# Autodesk Inventor assembly: V2-Output-.5inHex
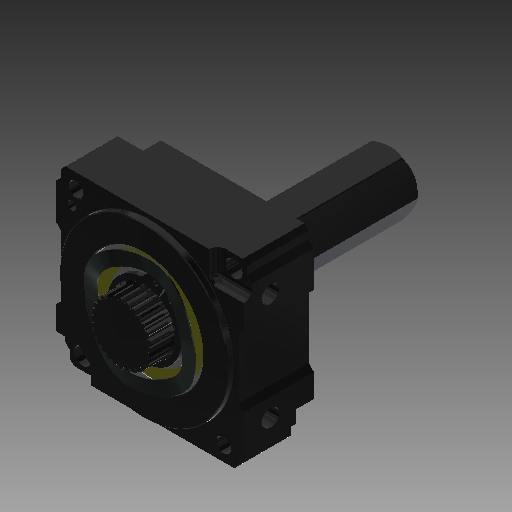
[picture p0: Inventor's stored thumbnail of the model, 512x512]
Saved by Autodesk Inventor 2023 (Build 270158000, 158)
## iProperties
Created: 2018-08-19
Part Number: V2-Output-.5inHex
Document SubType Name: Assembly
Mass: 68.0389 g
Surface Area: 166.113 cm^2
Volume: 34.5687 cm^3
Density: 1.96822 g/cm^3
## Documents named in this file (19)
- E:\Collaborative Robots\Collaborative Part Library\General Gearboxes\Planetaries\DEPRECATED Versaplanetary\V2 Stages\V2 Output Stage.iam
- E:\Collaborative Robots\Collaborative Part Library\General Gearboxes\Planetaries\DEPRECATED Versaplanetary\V2 Stages\V2 Output Housing.ipt
- E:\Collaborative Robots\Collaborative Part Library\General Gearboxes\Planetaries\DEPRECATED Versaplanetary\V2 Stages\Wave Washer.ipt
- E:\Collaborative Robots\Collaborative Part Library\General Gearboxes\Planetaries\DEPRECATED Versaplanetary\Output Shafts\VP 1-2inHex Output.ipt
- E:\Collaborative Robots\Collaborative Part Library\General Gearboxes\Planetaries\DEPRECATED Versaplanetary\V2 Stages\Retaining Ring.ipt
- E:\Collaborative Robots\Collaborative Part Library\General Gearboxes\Planetaries\DEPRECATED Versaplanetary\Output Shafts\VP 1-2inRound Output.ipt
- E:\Collaborative Robots\Collaborative Part Library\General Gearboxes\Planetaries\DEPRECATED Versaplanetary\Output Shafts\VP 3-8inHex Output.ipt
- E:\Collaborative Robots\Collaborative Part Library\General Gearboxes\Planetaries\DEPRECATED Versaplanetary\Output Shafts\VP CIM Output.ipt
- E:\Collaborative Robots\Collaborative Part Library\General Gearboxes\Planetaries\DEPRECATED Versaplanetary\Output Shafts\Universal Output shaft.ipt
- E:\Collaborative Robots\Collaborative Part Library\Power Transfer\Bearings and Bushings\Bearings\6902ZZ.ipt
- E:\Elipse 6814\Elipse Parts Library\Shaft Accessories\Bearings.ipt
- E:\Collaborative Robots\Collaborative Part Library\General Gearboxes\Planetaries\DEPRECATED Versaplanetary\VP 90 deg.ipt
- E:\Collaborative Robots\Collaborative Part Library\General Gearboxes\Planetaries\DEPRECATED Versaplanetary\Female Outputs\Universal Female Output Shaft 1_2_ Hex.ipt
- V2 Output Stage 90 deg.iam
- VP V2 Output Stage 1-2in Hex.iam
- VP V2 Output Stage 3-8in Hex.iam
- VP V2 Output Stage CIM.iam
- VP V2 Output Stage Female.iam
- VP V2 Output Stage Round.iam
## Components (12 placed, 11 different names)
1. V2 Output Housing:1 — Insert:2, Mate:2, Insert:18, Mate:3, Angle:6, Flush:7
2. 6902ZZ:1 — Insert:2, Insert:23
3. 6902ZZ:2 — Insert:18, Insert:19, Insert:20, Insert:22, Insert:24, Insert:25
4. Wave Washer:1 — Mate:2
5. Retaining Ring:1 — Angle:1, Angle:2, Angle:3, Angle:4, Angle:5, Insert:23
6. VP 1-2inHex Output:1 — Angle:1, Insert:20
7. VP 1-2inRound Output:1 — Angle:2, Insert:19
8. VP 3-8inHex Output:1 — Angle:3, Insert:22
9. VP CIM Output:1 — Angle:4, Insert:24
10. Universal Output shaft:1 — Angle:5, Insert:25, Insert:26
11. VP 90 deg:1 — Flush:8, Mate:5, Angle:7
12. Universal Female Output Shaft 1_2_ Hex:1 — Insert:26
## Relationships (21: Insert 9, Angle 7, Mate 3, Flush 2)
- Insert:2: V2 Output Housing:1 ↔ 6902ZZ:1
- Mate:2: V2 Output Housing:1 ↔ Wave Washer:1
- Angle:1 (0 deg): Retaining Ring:1 ↔ VP 1-2inHex Output:1
- Angle:2 (0 deg): Retaining Ring:1 ↔ VP 1-2inRound Output:1
- Angle:3 (0 deg): Retaining Ring:1 ↔ VP 3-8inHex Output:1
- Angle:4 (0 deg): Retaining Ring:1 ↔ VP CIM Output:1
- Angle:5 (0 deg): Retaining Ring:1 ↔ Universal Output shaft:1
- Insert:18: V2 Output Housing:1 ↔ 6902ZZ:2
- Insert:19: 6902ZZ:2 ↔ VP 1-2inRound Output:1
- Insert:20: 6902ZZ:2 ↔ VP 1-2inHex Output:1
- Insert:22: 6902ZZ:2 ↔ VP 3-8inHex Output:1
- Insert:23 (0.508 mm): 6902ZZ:1 ↔ Retaining Ring:1
- Insert:24: 6902ZZ:2 ↔ VP CIM Output:1
- Insert:25: 6902ZZ:2 ↔ Universal Output shaft:1
- Mate:3: V2 Output Housing:1
- Angle:6 (0 deg): V2 Output Housing:1
- Flush:8: VP 90 deg:1
- Mate:5: VP 90 deg:1
- Angle:7 (0 deg): VP 90 deg:1
- Flush:7: V2 Output Housing:1
- Insert:26: Universal Output shaft:1 ↔ Universal Female Output Shaft 1_2_ Hex:1
